# Autodesk Inventor assembly: gusset_mirrored
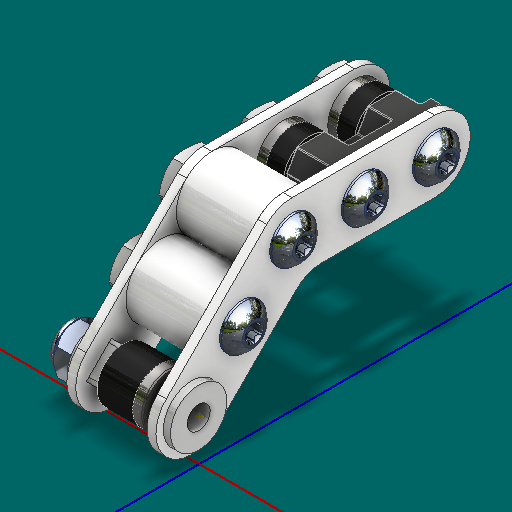
[picture p0: Inventor's stored thumbnail of the model, 512x512]
Saved by Autodesk Inventor 2025 (Build 290162000, 162)
## iProperties
Created: 2024-08-18
Part Number: gusset_mirrored
Document SubType Name: Assembly
Designer: averey
Author: averey
## Documents named in this file (17)
- C:\Users\avere\vex_robotics_high_stakes\hardware\cad\ATLAS\intake\first_stage\arm\gusset_mirrored\gusset_mirrored.iam
- C:\Users\avere\vex_robotics_high_stakes\hardware\cad\ATLAS\intake\first_stage\arm\gusset_mirrored\gusset_mirrored.ipt
- C:\Users\avere\vex_robotics_high_stakes\hardware\cad\VEX-CAD-Inventor\Motion\Spacers\Spacer Nylon .500 OD\NSpacer White .500 OD x .500.ipt
- C:\Users\avere\vex_robotics_high_stakes\hardware\cad\VEX-CAD-Inventor\Motion\Spacers\Spacer Nylon .500 OD.ipt
- C:\Users\avere\vex_robotics_high_stakes\hardware\cad\ATLAS\intake\first_stage\arm\gusset_mirrored\Insert Circle_mirrored.ipt
- C:\Users\avere\vex_robotics_high_stakes\hardware\cad\VEX-CAD-Inventor\Motion\Spacers\Washer Steel\SWasher .375 OD x .062500.ipt
- C:\Users\avere\vex_robotics_high_stakes\hardware\cad\VEX-CAD-Inventor\Motion\Spacers\Washer Steel.ipt
- C:\Users\avere\vex_robotics_high_stakes\hardware\cad\VEX-CAD-Inventor\Motion\Spacers\Spacer Nylon .375 OD\NSpacer .375 OD x .250.ipt
- C:\Users\avere\vex_robotics_high_stakes\hardware\cad\VEX-CAD-Inventor\Motion\Spacers\Spacer Nylon .375 OD.ipt
- C:\Users\avere\vex_robotics_high_stakes\hardware\cad\VEX-CAD-Inventor\Motion\Spacers\Washer Steel\SWasher .375 OD x .015625.ipt
- C:\Users\avere\vex_robotics_high_stakes\hardware\cad\VEX-CAD-Inventor\Structure\Hardware\Screw Steel - Star\SScrew Star Smooth .750.ipt
- C:\Users\avere\vex_robotics_high_stakes\hardware\cad\VEX-CAD-Inventor\Structure\Hardware\Screw Steel - Star.ipt
- C:\Users\avere\vex_robotics_high_stakes\hardware\cad\ATLAS\intake\first_stage\arm\gusset_mirrored\Bearing Flat Low Profile 2-Hole_mirrored.ipt
- C:\Users\avere\vex_robotics_high_stakes\hardware\cad\VEX-CAD-Inventor\Motion\Spacers\Spacer Nylon .375 OD\NSpacer .375 OD x .125.ipt
- C:\Users\avere\vex_robotics_high_stakes\hardware\cad\VEX-CAD-Inventor\Structure\Hardware\Nut Nylon\Nut Nylon - White.ipt
- C:\Users\avere\vex_robotics_high_stakes\hardware\cad\VEX-CAD-Inventor\Structure\Hardware\Nut Nylon.ipt
- C:\Users\avere\vex_robotics_high_stakes\hardware\cad\VEX-CAD-Inventor\Structure\Hardware\Nut Thin Nylock.ipt
## Components (23 placed, 11 different names)
1. gusset_mirrored:1 — Mate:1, Insert:1, Insert:2, Insert:3, Insert:4, Mate:3, Insert:11, Insert:12, Insert:18, Insert:20
2. gusset_mirrored:2 — Mate:1, Insert:1, Insert:5, Mate:2, Insert:6, Insert:7, Insert:16, Insert:15
3. NSpacer White .500 OD x .500:1 — Insert:2
4. NSpacer White .500 OD x .500:2 — Insert:3
5. Insert Circle_mirrored:1 — Mate:5, Insert:4, Mate:3
6. Insert Circle_mirrored:2 — Insert:5, Mate:2, Insert:10, Insert:22
7. SWasher .375 OD x .062500:1 — Insert:6, Insert:14
8. SWasher .375 OD x .062500:2 — Insert:7, Insert:13
9. NSpacer .375 OD x .250:1 — Insert:10, Insert:9
10. SWasher .375 OD x .015625:3 — Insert:8
11. SWasher .375 OD x .062500:4 — Insert:9, Insert:8
12. SScrew Star Smooth .750:1 — Insert:11
13. SScrew Star Smooth .750:2 — Insert:12
14. Bearing Flat Low Profile 2-Hole_mirrored:1 — Insert:21
15. NSpacer .375 OD x .125:2 — Insert:14
16. NSpacer .375 OD x .125:3 — Insert:21, Insert:13
17. Nut Nylon - White:1 — Insert:16
18. Nut Nylon - White:2 — Insert:15
19. SScrew Star Smooth .750:3 — Insert:18, Insert:17
20. Nut Nylon - White:3 — Insert:17
21. SScrew Star Smooth .750:4 — Insert:20, Insert:19
22. Nut Nylon - White:4 — Insert:19
23. Nut Thin Nylock:1 — Insert:22
## Relationships (26: Insert 22, Mate 4)
- Mate:1: gusset_mirrored:1 ↔ gusset_mirrored:2
- Insert:1 (12.7 mm): gusset_mirrored:1 ↔ gusset_mirrored:2
- Insert:2: gusset_mirrored:1 ↔ NSpacer White .500 OD x .500:1
- Insert:3: gusset_mirrored:1 ↔ NSpacer White .500 OD x .500:2
- Mate:5: Insert Circle_mirrored:1
- Insert:4: gusset_mirrored:1 ↔ Insert Circle_mirrored:1
- Mate:3: gusset_mirrored:1 ↔ Insert Circle_mirrored:1
- Insert:5: gusset_mirrored:2 ↔ Insert Circle_mirrored:2
- Mate:2: gusset_mirrored:2 ↔ Insert Circle_mirrored:2
- Insert:6: gusset_mirrored:2 ↔ SWasher .375 OD x .062500:1
- Insert:7: gusset_mirrored:2 ↔ SWasher .375 OD x .062500:2
- Insert:10: Insert Circle_mirrored:2 ↔ NSpacer .375 OD x .250:1
- Insert:9: NSpacer .375 OD x .250:1 ↔ SWasher .375 OD x .062500:4
- Insert:8: SWasher .375 OD x .015625:3 ↔ SWasher .375 OD x .062500:4
- Insert:11: gusset_mirrored:1 ↔ SScrew Star Smooth .750:1
- Insert:12: gusset_mirrored:1 ↔ SScrew Star Smooth .750:2
- Insert:14: SWasher .375 OD x .062500:1 ↔ NSpacer .375 OD x .125:2
- Insert:21 (1.27 mm): Bearing Flat Low Profile 2-Hole_mirrored:1 ↔ NSpacer .375 OD x .125:3
- Insert:13: SWasher .375 OD x .062500:2 ↔ NSpacer .375 OD x .125:3
- Insert:16: gusset_mirrored:2 ↔ Nut Nylon - White:1
- Insert:15: gusset_mirrored:2 ↔ Nut Nylon - White:2
- Insert:18: gusset_mirrored:1 ↔ SScrew Star Smooth .750:3
- Insert:17 (15.875 mm): SScrew Star Smooth .750:3 ↔ Nut Nylon - White:3
- Insert:20: gusset_mirrored:1 ↔ SScrew Star Smooth .750:4
- Insert:19 (15.875 mm): SScrew Star Smooth .750:4 ↔ Nut Nylon - White:4
- Insert:22: Insert Circle_mirrored:2 ↔ Nut Thin Nylock:1
